# Autodesk Inventor assembly: Module with Full Cover V1
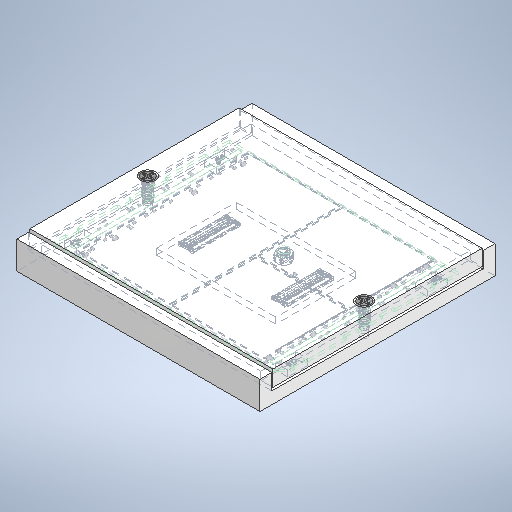
[picture p0: Inventor's stored thumbnail of the model, 512x512]
Saved by Autodesk Inventor 2025 (Build 290162000, 162)
## iProperties
Created: 2024-03-28
Part Number: Module with Full Cover V1
Document SubType Name: Assembly
Designer: cfang
Author: cfang
## Documents named in this file (6)
- C:\Users\cfang\Desktop\nebraska-silicon-lab\Hardware\ETL\Irradiation Fixture\Module with Full Cover V1.iam
- C:\Users\cfang\Desktop\nebraska-silicon-lab\Hardware\ETL\modules\tamale v1.5\Tamale - V1p5p2.iam
- C:\Users\cfang\Desktop\nebraska-silicon-lab\Hardware\ETL\Irradiation Fixture\Glass Slide Spacer V1.ipt
- C:\Users\cfang\Desktop\nebraska-silicon-lab\Hardware\ETL\Irradiation Fixture\91420A003_Steel Phillips Flat Head Screws\91420A003_Steel Phillips Flat Head Screws.ipt
- C:\Users\cfang\Desktop\nebraska-silicon-lab\Hardware\ETL\Irradiation Fixture\Module Holder Full V1.ipt
- C:\Users\cfang\Desktop\nebraska-silicon-lab\Hardware\ETL\Irradiation Fixture\Module Holder Full Cover V1.ipt
## Components (6 placed, 5 different names)
1. Tamale - V1p5p2:1 [sub-assembly] — Insert:1, Insert:2, Insert:3
2. Glass Slide Spacer V1:1
3. 91420A003_Steel Phillips Flat Head Screws:1 — Insert:5
4. Module Holder Full V1:1 — Insert:1, Insert:2
5. Module Holder Full Cover V1:1 — Insert:3, Insert:4, Insert:5
6. 91420A003_Steel Phillips Flat Head Screws:2 — Insert:4
## Relationships (8: Insert 5, Mate 2, Flush 1)
- [Mate]: Tamale - V1p5p2:1 ↔ Glass Slide Spacer V1:1
- [Flush]: Tamale - V1p5p2:1 ↔ Glass Slide Spacer V1:1
- [Mate] (0.6 mm): Tamale - V1p5p2:1 ↔ Glass Slide Spacer V1:1
- Insert:1: Tamale - V1p5p2:1 ↔ Module Holder Full V1:1
- Insert:2: Tamale - V1p5p2:1 ↔ Module Holder Full V1:1
- Insert:3: Tamale - V1p5p2:1 ↔ Module Holder Full Cover V1:1
- Insert:4: Module Holder Full Cover V1:1 ↔ 91420A003_Steel Phillips Flat Head Screws:2
- Insert:5: 91420A003_Steel Phillips Flat Head Screws:1 ↔ Module Holder Full Cover V1:1
## Named parameters: d3_d5 = 0.6 mm
